# Autodesk Inventor assembly: Sestava1
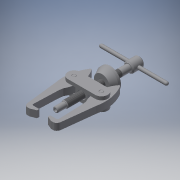
[picture p0: Inventor's stored thumbnail of the model, 180x180]
Saved by Autodesk Inventor 2019 (Build 230136000, 136)
## iProperties
Created: 2020-02-04
Part Number: Sestava1
Material: Všeobecné
Document SubType Name: Assembly
Designer: hynek
Author: hynek
## Documents named in this file (7)
- C:\Kyberna prvák\TEK\Sestava1.iam
- C:\Kyberna prvák\TEK\Součást25.ipt
- C:\Kyberna prvák\TEK\Součást21.ipt
- C:\Kyberna prvák\TEK\teleso.ipt
- C:\Kyberna prvák\TEK\Součást26.ipt
- C:\Kyberna prvák\TEK\Součást23.ipt
- C:\Kyberna prvák\TEK\tyc.ipt
## Components (8 placed, 6 different names)
1. Součást25:1 — Proti sobě:1, Proti sobě:2, Proti sobě:3, Proti sobě:4, Úhel:1, Proti sobě:5, Proti sobě:6, Vložit:1, Proti sobě:9, Proti sobě:10, Proti sobě:11, Proti sobě:12, Proti sobě:13, Proti sobě:14
2. Součást21:1 — Proti sobě:4, Úhel:1, Proti sobě:5
3. Součást21:2 — Proti sobě:6, Proti sobě:11, Proti sobě:12
4. teleso:1 — Vložit:1, Proti sobě:9
5. teleso:2 — Proti sobě:10, Proti sobě:19
6. Součást26:1 — Proti sobě:13, Proti sobě:14, Proti sobě:15, Proti sobě:16, Proti sobě:18, Proti sobě:19
7. Součást23:1 — Proti sobě:15, Proti sobě:18
8. tyc:1 — Proti sobě:16, Proti sobě:17
## Relationships (19: Mate 17, Angle 1, Insert 1)
- Proti sobě:1 [Mate]: Součást25:1
- Proti sobě:2 [Mate]: Součást25:1
- Proti sobě:3 [Mate]: Součást25:1
- Proti sobě:4 [Mate]: Součást25:1 ↔ Součást21:1
- Úhel:1 [Angle] (0 deg): Součást25:1 ↔ Součást21:1
- Proti sobě:5 [Mate]: Součást25:1 ↔ Součást21:1
- Proti sobě:6 [Mate]: Součást25:1 ↔ Součást21:2
- Vložit:1 [Insert]: Součást25:1 ↔ teleso:1
- Proti sobě:9 [Mate]: Součást25:1 ↔ teleso:1
- Proti sobě:10 [Mate]: Součást25:1 ↔ teleso:2
- Proti sobě:11 [Mate]: Součást25:1 ↔ Součást21:2
- Proti sobě:12 [Mate]: Součást25:1 ↔ Součást21:2
- Proti sobě:13 [Mate]: Součást25:1 ↔ Součást26:1
- Proti sobě:14 [Mate]: Součást25:1 ↔ Součást26:1
- Proti sobě:15 [Mate]: Součást26:1 ↔ Součást23:1
- Proti sobě:16 [Mate]: Součást26:1 ↔ tyc:1
- Proti sobě:17 [Mate]: tyc:1
- Proti sobě:18 [Mate] (-15 mm): Součást26:1 ↔ Součást23:1
- Proti sobě:19 [Mate] (-40 mm): teleso:2 ↔ Součást26:1
